# Autodesk Inventor assembly: whole_assembly
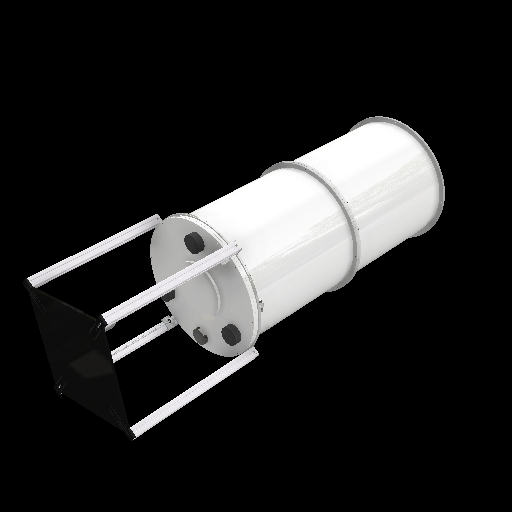
[picture p0: Inventor's stored thumbnail of the model, 512x512]
Saved by Autodesk Inventor 2026.1 (Build 301233000, 233)
## iProperties
Created: 2025-09-18
Part Number: whole_assembly
Document SubType Name: Assembly
Designer: drago
Author: drago
## Documents named in this file (3)
- C:\Users\drago\Desktop\_QIST4500_Multidisciplinary_Team_Project\Proteox MX magnet positioner CAD\whole_assembly.iam
- C:\Users\drago\Desktop\_QIST4500_Multidisciplinary_Team_Project\Proteox MX magnet positioner CAD\proteox_fridge.iam
- C:\Users\drago\Desktop\_QIST4500_Multidisciplinary_Team_Project\Proteox MX magnet positioner CAD\gantry_frame.iam
## Components (2 placed, 2 different names)
1. proteox_fridge:1 [sub-assembly] — Mate:1, Mate:3, Mate:4
2. gantry_frame:1 [sub-assembly] — Mate:2, Angle:1, Mate:4
## Relationships (5: Mate 4, Angle 1)
- Mate:1: proteox_fridge:1
- Mate:2: gantry_frame:1
- Mate:3: proteox_fridge:1
- Angle:1 (11.25 deg): gantry_frame:1
- Mate:4: proteox_fridge:1 ↔ gantry_frame:1
